# Autodesk Inventor assembly: XCarriage
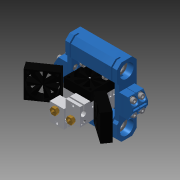
[picture p0: Inventor's stored thumbnail of the model, 180x180]
Saved by Autodesk Inventor 2015 SP1 (Build 190203100, 203)
## iProperties
Created: 2014-12-10
Part Number: XCarriage
Document SubType Name: Assembly
Designer: Jack
Mass: 269.669 g
Surface Area: 979.869 cm^2
Volume: 134.924 cm^3
Density: 1.99868 g/cm^3
Author: Jack
Title: X Carriage
## Documents named in this file (11)
- C:\Users\Jack\ownCloud\Projects\CrossBot\InventorModel\XAxis\XCarriage.iam
- C:\Users\Jack\ownCloud\Projects\CrossBot\InventorModel\HotEnds\E3DChimera\E3DChimera.iam
- C:\Users\Jack\ownCloud\Projects\CrossBot\InventorModel\Electronics\EndStops\EndStopOptical.ipt
- C:\Users\Jack\ownCloud\Projects\CrossBot\InventorModel\XAxis\XCarriageBeltClipRound.ipt
- C:\Users\Jack\ownCloud\Projects\CrossBot\InventorModel\Hardware\Nuts\Nut3.ipt
- C:\Users\Jack\ownCloud\Projects\CrossBot\InventorModel\Hardware\BoltWashers\BoltWasher3\BoltWasher3x16.iam
- C:\Users\Jack\ownCloud\Projects\CrossBot\InventorModel\Hardware\Bolts\SHCS\SHCS3\SHCS3x8.ipt
- C:\Users\Jack\ownCloud\Projects\CrossBot\InventorModel\XAxis\ChimeraXCarriage5.ipt
- C:\Users\Jack\ownCloud\Projects\CrossBot\InventorModel\Hardware\Bolts\SHCS\SHCS3\SHCS3x18.ipt
- C:\Users\Jack\ownCloud\Projects\CrossBot\InventorModel\Hardware\Bearing\BearingLinear\BearingLinearLMUW8.ipt
- C:\Users\Jack\ownCloud\Projects\CrossBot\InventorModel\HotEnds\E3DChimera\Fan30mm.ipt
## Components (39 placed, 10 different names)
1. E3DChimera:1 [sub-assembly] — Mate:91, Mate:92, Mate:93, Mate:94
2. EndStopOptical:1 — Mate:84, Mate:85, Mate:86, Mate:87, Mate:155
3. XCarriageBeltClipRound:1 — Mate:41, Mate:43, Mate:53, Mate:56, Mate:136
4. XCarriageBeltClipRound:2 — Mate:42, Mate:44, Mate:54, Mate:55, Mate:135
5. XCarriageBeltClipRound:3 — Mate:45, Mate:47, Mate:49, Mate:51, Mate:149
6. XCarriageBeltClipRound:4 — Mate:46, Mate:48, Mate:50, Mate:52, Mate:150
7. Nut3:15 — Mate:89
8. Nut3:16 — Mate:88
9. SHCS3x8:1 — Mate:84, Mate:85, Mate:89, Mate:154
10. SHCS3x8:2 — Mate:86, Mate:87, Mate:88, Mate:153
11. ChimeraXCarriage5:1 — Mate:91, Mate:92, Mate:93, Mate:94, Angle:1, Angle:2, Angle:3, Angle:4, Mate:107, Mate:108, Mate:109, Mate:110, Mate:111, Mate:112, Mate:113, Mate:114, Mate:115, Mate:116, Mate:117, Mate:118, Mate:123, Mate:124, Mate:125, Mate:126, Mate:131, Mate:132, Mate:133, Mate:134, Mate:135, Mate:136, Mate:137, Mate:138, Mate:139, Mate:140, Mate:145, Mate:146, Mate:147, Mate:148, Mate:149, Mate:150, Mate:151, Flush:6, Mate:152, Flush:7, Angle:5, Mate:153, Mate:154, Mate:155
12. SHCS3x18:1 — Mate:113, Mate:118, Mate:120
13. SHCS3x18:2 — Mate:112, Mate:115, Mate:122
14. SHCS3x18:3 — Mate:114, Mate:117, Mate:119
15. SHCS3x18:4 — Mate:111, Mate:116, Mate:121
16. BearingLinearLMUW8:1 — Mate:151, Flush:6
17. BearingLinearLMUW8:2 — Mate:152, Flush:7
18. Fan30mm:1 — Angle:5
19. Fan30mm:2
20. Nut3:13 — Angle:4, Mate:107, Mate:122
21. Nut3:12 — Angle:3, Mate:110, Mate:121
22. Nut3:10 — Angle:1, Mate:109, Mate:119
23. Nut3:9 — Angle:2, Mate:108, Mate:120
24. BoltWasher3x16:1 [sub-assembly] — Mate:42, Mate:55, Mate:124, Mate:130
25. BoltWasher3x16:2 [sub-assembly] — Mate:41, Mate:56, Mate:126, Mate:128
26. BoltWasher3x16:3 [sub-assembly] — Mate:43, Mate:53, Mate:125, Mate:127
27. BoltWasher3x16:4 [sub-assembly] — Mate:44, Mate:54, Mate:123, Mate:129
28. BoltWasher3x16:5 [sub-assembly] — Mate:45, Mate:49, Mate:142, Mate:148
29. BoltWasher3x16:6 [sub-assembly] — Mate:46, Mate:50, Mate:144, Mate:145
30. BoltWasher3x16:7 [sub-assembly] — Mate:47, Mate:51, Mate:141, Mate:147
31. BoltWasher3x16:8 [sub-assembly] — Mate:48, Mate:52, Mate:143, Mate:146
32. Nut3:1 — Mate:139, Mate:141
33. Nut3:2 — Mate:137, Mate:143
34. Nut3:3 — Mate:127, Mate:134
35. Nut3:4 — Mate:129, Mate:133
36. Nut3:5 — Mate:140, Mate:142
37. Nut3:6 — Mate:138, Mate:144
38. Nut3:7 — Mate:128, Mate:132
39. Nut3:8 — Mate:130, Mate:131
## Relationships (82: Mate 75, Angle 5, Flush 2)
- Mate:41: XCarriageBeltClipRound:1 ↔ BoltWasher3x16:2
- Mate:42: XCarriageBeltClipRound:2 ↔ BoltWasher3x16:1
- Mate:43: XCarriageBeltClipRound:1 ↔ BoltWasher3x16:3
- Mate:44: XCarriageBeltClipRound:2 ↔ BoltWasher3x16:4
- Mate:45: XCarriageBeltClipRound:3 ↔ BoltWasher3x16:5
- Mate:46: XCarriageBeltClipRound:4 ↔ BoltWasher3x16:6
- Mate:47: XCarriageBeltClipRound:3 ↔ BoltWasher3x16:7
- Mate:48: XCarriageBeltClipRound:4 ↔ BoltWasher3x16:8
- Mate:49: XCarriageBeltClipRound:3 ↔ BoltWasher3x16:5
- Mate:50: XCarriageBeltClipRound:4 ↔ BoltWasher3x16:6
- Mate:51: XCarriageBeltClipRound:3 ↔ BoltWasher3x16:7
- Mate:52: XCarriageBeltClipRound:4 ↔ BoltWasher3x16:8
- Mate:53: XCarriageBeltClipRound:1 ↔ BoltWasher3x16:3
- Mate:54: XCarriageBeltClipRound:2 ↔ BoltWasher3x16:4
- Mate:55: XCarriageBeltClipRound:2 ↔ BoltWasher3x16:1
- Mate:56: XCarriageBeltClipRound:1 ↔ BoltWasher3x16:2
- Mate:84: EndStopOptical:1 ↔ SHCS3x8:1
- Mate:85: EndStopOptical:1 ↔ SHCS3x8:1
- Mate:86: EndStopOptical:1 ↔ SHCS3x8:2
- Mate:87: EndStopOptical:1 ↔ SHCS3x8:2
- Mate:88: Nut3:16 ↔ SHCS3x8:2
- Mate:89: Nut3:15 ↔ SHCS3x8:1
- Mate:91: E3DChimera:1 ↔ ChimeraXCarriage5:1
- Mate:92: E3DChimera:1 ↔ ChimeraXCarriage5:1
- Mate:93: E3DChimera:1 ↔ ChimeraXCarriage5:1
- Mate:94: E3DChimera:1 ↔ ChimeraXCarriage5:1
- Angle:1 (0 deg): ChimeraXCarriage5:1 ↔ Nut3:10
- Angle:2 (0 deg): ChimeraXCarriage5:1 ↔ Nut3:9
- Angle:3 (0 deg): ChimeraXCarriage5:1 ↔ Nut3:12
- Angle:4 (0 deg): ChimeraXCarriage5:1 ↔ Nut3:13
- Mate:107: ChimeraXCarriage5:1 ↔ Nut3:13
- Mate:108: ChimeraXCarriage5:1 ↔ Nut3:9
- Mate:109: ChimeraXCarriage5:1 ↔ Nut3:10
- Mate:110: ChimeraXCarriage5:1 ↔ Nut3:12
- Mate:111: ChimeraXCarriage5:1 ↔ SHCS3x18:4
- Mate:112: ChimeraXCarriage5:1 ↔ SHCS3x18:2
- Mate:113: ChimeraXCarriage5:1 ↔ SHCS3x18:1
- Mate:114: ChimeraXCarriage5:1 ↔ SHCS3x18:3
- Mate:115: ChimeraXCarriage5:1 ↔ SHCS3x18:2
- Mate:116: ChimeraXCarriage5:1 ↔ SHCS3x18:4
- Mate:117: ChimeraXCarriage5:1 ↔ SHCS3x18:3
- Mate:118: ChimeraXCarriage5:1 ↔ SHCS3x18:1
- Mate:119: SHCS3x18:3 ↔ Nut3:10
- Mate:120: SHCS3x18:1 ↔ Nut3:9
- Mate:121: SHCS3x18:4 ↔ Nut3:12
- Mate:122: SHCS3x18:2 ↔ Nut3:13
- Mate:123: ChimeraXCarriage5:1 ↔ BoltWasher3x16:4
- Mate:124: ChimeraXCarriage5:1 ↔ BoltWasher3x16:1
- Mate:125: ChimeraXCarriage5:1 ↔ BoltWasher3x16:3
- Mate:126: ChimeraXCarriage5:1 ↔ BoltWasher3x16:2
- Mate:127: BoltWasher3x16:3 ↔ Nut3:3
- Mate:128: BoltWasher3x16:2 ↔ Nut3:7
- Mate:129: BoltWasher3x16:4 ↔ Nut3:4
- Mate:130: BoltWasher3x16:1 ↔ Nut3:8
- Mate:131: ChimeraXCarriage5:1 ↔ Nut3:8
- Mate:132: ChimeraXCarriage5:1 ↔ Nut3:7
- Mate:133: ChimeraXCarriage5:1 ↔ Nut3:4
- Mate:134: ChimeraXCarriage5:1 ↔ Nut3:3
- Mate:135: XCarriageBeltClipRound:2 ↔ ChimeraXCarriage5:1
- Mate:136: XCarriageBeltClipRound:1 ↔ ChimeraXCarriage5:1
- Mate:137: ChimeraXCarriage5:1 ↔ Nut3:2
- Mate:138: ChimeraXCarriage5:1 ↔ Nut3:6
- Mate:139: ChimeraXCarriage5:1 ↔ Nut3:1
- Mate:140: ChimeraXCarriage5:1 ↔ Nut3:5
- Mate:141: BoltWasher3x16:7 ↔ Nut3:1
- Mate:142: BoltWasher3x16:5 ↔ Nut3:5
- Mate:143: BoltWasher3x16:8 ↔ Nut3:2
- Mate:144: BoltWasher3x16:6 ↔ Nut3:6
- Mate:145: ChimeraXCarriage5:1 ↔ BoltWasher3x16:6
- Mate:146: ChimeraXCarriage5:1 ↔ BoltWasher3x16:8
- Mate:147: ChimeraXCarriage5:1 ↔ BoltWasher3x16:7
- Mate:148: ChimeraXCarriage5:1 ↔ BoltWasher3x16:5
- Mate:149: XCarriageBeltClipRound:3 ↔ ChimeraXCarriage5:1
- Mate:150: XCarriageBeltClipRound:4 ↔ ChimeraXCarriage5:1
- Mate:151: ChimeraXCarriage5:1 ↔ BearingLinearLMUW8:1
- Flush:6: ChimeraXCarriage5:1 ↔ BearingLinearLMUW8:1
- Mate:152: ChimeraXCarriage5:1 ↔ BearingLinearLMUW8:2
- Flush:7: ChimeraXCarriage5:1 ↔ BearingLinearLMUW8:2
- Angle:5 (0 deg): ChimeraXCarriage5:1 ↔ Fan30mm:1
- Mate:153: SHCS3x8:2 ↔ ChimeraXCarriage5:1
- Mate:154: SHCS3x8:1 ↔ ChimeraXCarriage5:1
- Mate:155: EndStopOptical:1 ↔ ChimeraXCarriage5:1
